# Autodesk Inventor assembly: ASY МОО 060 ракета
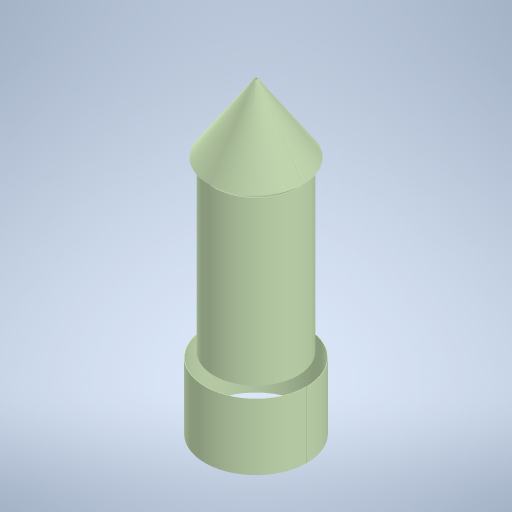
[picture p0: Inventor's stored thumbnail of the model, 512x512]
Saved by Autodesk Inventor 2024.2 (Build 282272000, 272)
## iProperties
Created: 2024-05-19
Part Number: ASY МОО 060 ракета
Document SubType Name: Assembly
Designer: admin
Author: admin
## Documents named in this file (5)
- C:\Users\admin\Documents\Inventor\Manturovo\отстойник осветлитель\ASY МОО 060 ракета.iam
- C:\Users\admin\Documents\Inventor\Manturovo\отстойник осветлитель\МОО DIM 061  ракета.ipt
- C:\Users\admin\Documents\Inventor\Manturovo\отстойник осветлитель\ракета\МОО 061 ракета хвост.ipt
- C:\Users\admin\Documents\Inventor\Manturovo\отстойник осветлитель\ракета\МОО 062 ракета тело.ipt
- C:\Users\admin\Documents\Inventor\Manturovo\отстойник осветлитель\ракета\МОО 063 ракета нос.ipt
## Components (4 placed, 4 different names)
1. МОО DIM 061  ракета:1
2. МОО 061 ракета хвост:1 — Rigid:1, Mate:2
3. МОО 062 ракета тело:1 — Rigid:1, Rigid:2
4. МОО 063 ракета нос:1 — Rigid:2
## Relationships (3: WeldJoint 2, Mate 1)
- Rigid:1 [WeldJoint] (10 mm): МОО 061 ракета хвост:1 ↔ МОО 062 ракета тело:1
- Rigid:2 [WeldJoint] (10 mm): МОО 062 ракета тело:1 ↔ МОО 063 ракета нос:1
- Mate:2: МОО 061 ракета хвост:1
